# Autodesk Inventor assembly: Mellie Cart Wheel Mount
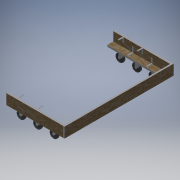
[picture p0: Inventor's stored thumbnail of the model, 180x180]
Saved by Autodesk Inventor 2018.2 (Build 222227000, 227)
## iProperties
Created: 2018-02-21
Part Number: Mellie Cart Wheel Mount
Document SubType Name: Assembly
Designer: owner
Author: owner
## Documents named in this file (7)
- Z:\The Pickle - 4 - Copy\Final Carts\Mellie Cart\Mellie Cart Wheel Mount.iam
- Z:\The Pickle - 4 - Copy\Final Carts\Stuff Used By All Carts\WHEELS.ipt
- Z:\The Pickle - 4 - Copy\Final Carts\Mellie Cart\Mellie Wheel Mount Plywood Side.ipt
- Z:\The Pickle - 4 - Copy\Final Carts\Mellie Cart\Mellie Wheel Mount Plywood Bottom.ipt
- Z:\The Pickle - 4 - Copy\Final Carts\Locking Mech\Plywood Pickle Mount Corner Bracket.ipt
- Z:\The Pickle - 4 - Copy\Final Carts\Locking Mech\Plywood Pickle Mount Triangle Bracket.ipt
- Z:\The Pickle - 4 - Copy\Final Carts\Mellie Cart\Mellie Wheel Mount Plywood Front.ipt
## Components (21 placed, 6 different names)
1. Mellie Wheel Mount Plywood Side:1 — Mate:1, Flush:8, Mate:3, Mate:6, Mate:7, Mate:10, Mate:11, Flush:14, Mate:23, Flush:21, Flush:35
2. Mellie Wheel Mount Plywood Bottom:1 — Mate:1, Mate:2, Mate:4, Mate:5, Flush:30, Mate:31
3. WHEELS:1 — Flush:24, Flush:27, Flush:31, Mate:29, Flush:32
4. WHEELS:2 — Flush:23, Flush:28, Flush:34
5. WHEELS:3 — Flush:22, Flush:23, Flush:28, Flush:29, Flush:33
6. WHEELS:4 — Flush:24, Flush:25, Flush:26, Mate:29, Mate:30, Flush:33
7. WHEELS:5 — Flush:25, Flush:26, Flush:27, Mate:27, Mate:30, Flush:34
8. WHEELS:6 — Flush:22, Flush:29, Flush:30, Flush:32, Mate:31
9. Plywood Pickle Mount Corner Bracket:1 — Mate:4, Mate:10, Flush:18, Mate:26
10. Plywood Pickle Mount Triangle Bracket:1 — Flush:8, Mate:2, Mate:3
11. Plywood Pickle Mount Corner Bracket:2 — Mate:6, Flush:17, Mate:25, Mate:26
12. Plywood Pickle Mount Corner Bracket:5 — Mate:18, Mate:20, Flush:18
13. Plywood Pickle Mount Corner Bracket:6 — Mate:17, Flush:13, Flush:17
14. Plywood Pickle Mount Corner Bracket:7 — Mate:16, Mate:19, Flush:16
15. Plywood Pickle Mount Corner Bracket:8 — Mate:15, Flush:12, Flush:15
16. Plywood Pickle Mount Triangle Bracket:8 — Mate:13, Mate:14, Flush:11
17. Plywood Pickle Mount Corner Bracket:9 — Mate:7, Flush:15, Flush:21, Mate:24
18. Plywood Pickle Mount Corner Bracket:10 — Mate:5, Mate:11, Flush:16, Mate:24, Mate:25
19. Mellie Wheel Mount Plywood Bottom:2 — Mate:12, Flush:9, Flush:10, Mate:14, Mate:19, Mate:20, Flush:31, Mate:27
20. Mellie Wheel Mount Plywood Side:2 — Mate:12, Flush:9, Flush:10, Mate:13, Flush:11, Mate:15, Mate:16, Mate:17, Mate:18, Flush:12, Flush:13, Flush:14, Flush:36
21. Mellie Wheel Mount Plywood Front:1 — Mate:23, Flush:35, Flush:36
## Relationships (53: Flush 27, Mate 26)
- Mate:1: Mellie Wheel Mount Plywood Side:1 ↔ Mellie Wheel Mount Plywood Bottom:1
- Flush:8: Mellie Wheel Mount Plywood Side:1 ↔ Plywood Pickle Mount Triangle Bracket:1
- Mate:2: Mellie Wheel Mount Plywood Bottom:1 ↔ Plywood Pickle Mount Triangle Bracket:1
- Mate:3: Mellie Wheel Mount Plywood Side:1 ↔ Plywood Pickle Mount Triangle Bracket:1
- Mate:4: Mellie Wheel Mount Plywood Bottom:1 ↔ Plywood Pickle Mount Corner Bracket:1
- Mate:5: Mellie Wheel Mount Plywood Bottom:1 ↔ Plywood Pickle Mount Corner Bracket:10
- Mate:6: Mellie Wheel Mount Plywood Side:1 ↔ Plywood Pickle Mount Corner Bracket:2
- Mate:7: Mellie Wheel Mount Plywood Side:1 ↔ Plywood Pickle Mount Corner Bracket:9
- Mate:10: Mellie Wheel Mount Plywood Side:1 ↔ Plywood Pickle Mount Corner Bracket:1
- Mate:11: Mellie Wheel Mount Plywood Side:1 ↔ Plywood Pickle Mount Corner Bracket:10
- Mate:12: Mellie Wheel Mount Plywood Bottom:2 ↔ Mellie Wheel Mount Plywood Side:2
- Flush:9: Mellie Wheel Mount Plywood Bottom:2 ↔ Mellie Wheel Mount Plywood Side:2
- Flush:10: Mellie Wheel Mount Plywood Bottom:2 ↔ Mellie Wheel Mount Plywood Side:2
- Mate:13: Plywood Pickle Mount Triangle Bracket:8 ↔ Mellie Wheel Mount Plywood Side:2
- Mate:14: Plywood Pickle Mount Triangle Bracket:8 ↔ Mellie Wheel Mount Plywood Bottom:2
- Flush:11: Plywood Pickle Mount Triangle Bracket:8 ↔ Mellie Wheel Mount Plywood Side:2
- Mate:15: Plywood Pickle Mount Corner Bracket:8 ↔ Mellie Wheel Mount Plywood Side:2
- Mate:16: Plywood Pickle Mount Corner Bracket:7 ↔ Mellie Wheel Mount Plywood Side:2
- Mate:17: Plywood Pickle Mount Corner Bracket:6 ↔ Mellie Wheel Mount Plywood Side:2
- Mate:18: Plywood Pickle Mount Corner Bracket:5 ↔ Mellie Wheel Mount Plywood Side:2
- Flush:12: Plywood Pickle Mount Corner Bracket:8 ↔ Mellie Wheel Mount Plywood Side:2
- Flush:13: Plywood Pickle Mount Corner Bracket:6 ↔ Mellie Wheel Mount Plywood Side:2
- Mate:19: Plywood Pickle Mount Corner Bracket:7 ↔ Mellie Wheel Mount Plywood Bottom:2
- Mate:20: Plywood Pickle Mount Corner Bracket:5 ↔ Mellie Wheel Mount Plywood Bottom:2
- Flush:14: Mellie Wheel Mount Plywood Side:1 ↔ Mellie Wheel Mount Plywood Side:2
- Flush:15: Plywood Pickle Mount Corner Bracket:8 ↔ Plywood Pickle Mount Corner Bracket:9
- Flush:16: Plywood Pickle Mount Corner Bracket:7 ↔ Plywood Pickle Mount Corner Bracket:10
- Flush:17: Plywood Pickle Mount Corner Bracket:2 ↔ Plywood Pickle Mount Corner Bracket:6
- Flush:18: Plywood Pickle Mount Corner Bracket:1 ↔ Plywood Pickle Mount Corner Bracket:5
- Mate:23: Mellie Wheel Mount Plywood Side:1 ↔ Mellie Wheel Mount Plywood Front:1
- Flush:21 (114.3 mm): Mellie Wheel Mount Plywood Side:1 ↔ Plywood Pickle Mount Corner Bracket:9
- Mate:24 (101.6 mm): Plywood Pickle Mount Corner Bracket:9 ↔ Plywood Pickle Mount Corner Bracket:10
- Mate:25 (101.6 mm): Plywood Pickle Mount Corner Bracket:2 ↔ Plywood Pickle Mount Corner Bracket:10
- Mate:26 (101.6 mm): Plywood Pickle Mount Corner Bracket:1 ↔ Plywood Pickle Mount Corner Bracket:2
- Flush:22: WHEELS:3 ↔ WHEELS:6
- Flush:23: WHEELS:2 ↔ WHEELS:3
- Flush:24: WHEELS:1 ↔ WHEELS:4
- Flush:25: WHEELS:4 ↔ WHEELS:5
- Flush:26: WHEELS:4 ↔ WHEELS:5
- Flush:27: WHEELS:1 ↔ WHEELS:5
- Flush:28: WHEELS:2 ↔ WHEELS:3
- Flush:29: WHEELS:3 ↔ WHEELS:6
- Flush:30 (6.35 mm): Mellie Wheel Mount Plywood Bottom:1 ↔ WHEELS:6
- Flush:31 (6.35 mm): WHEELS:1 ↔ Mellie Wheel Mount Plywood Bottom:2
- Mate:27: WHEELS:5 ↔ Mellie Wheel Mount Plywood Bottom:2
- Mate:29 (107.7976 mm): WHEELS:1 ↔ WHEELS:4
- Mate:30 (107.7976 mm): WHEELS:4 ↔ WHEELS:5
- Flush:32: WHEELS:1 ↔ WHEELS:6
- Flush:33: WHEELS:3 ↔ WHEELS:4
- Flush:34: WHEELS:2 ↔ WHEELS:5
- Mate:31: Mellie Wheel Mount Plywood Bottom:1 ↔ WHEELS:6
- Flush:35: Mellie Wheel Mount Plywood Side:1 ↔ Mellie Wheel Mount Plywood Front:1
- Flush:36: Mellie Wheel Mount Plywood Side:2 ↔ Mellie Wheel Mount Plywood Front:1
